# Autodesk Inventor assembly: scaffolding
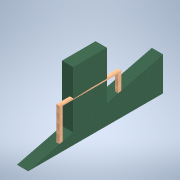
[picture p0: Inventor's stored thumbnail of the model, 180x180]
Saved by Autodesk Inventor 2020.2 (Build 242310000, 310)
## iProperties
Created: 2020-03-28
Part Number: scaffolding
Document SubType Name: Assembly
Designer: robst
Author: robst
## Documents named in this file (5)
- C:\git\CAD-Development\robSteele\HouseProjects\RoofChimney\scaffolding.iam
- C:\git\CAD-Development\robSteele\HouseProjects\RoofChimney\roof.ipt
- C:\git\CAD-Development\robSteele\HouseProjects\RoofChimney\4x4x18-post.ipt
- C:\git\CAD-Development\robSteele\HouseProjects\RoofChimney\2x4x66-board.ipt
- C:\git\CAD-Development\robSteele\HouseProjects\RoofChimney\4x4x33-5_8-post.ipt
## Components (4 placed, 4 different names)
1. roof:1 — Mate:1, Flush:1, Flush:2, Mate:3, Flush:5
2. 4x4x18-post:1 — Mate:1, Flush:1, Flush:2, Mate:2, Flush:3, Flush:4
3. 2x4x66-board:1 — Mate:2, Flush:3, Flush:4, Flush:6
4. 4x4x33-5_8-post:1 — Mate:3, Flush:5, Flush:6
## Relationships (9: Flush 6, Mate 3)
- Mate:1: roof:1 ↔ 4x4x18-post:1
- Flush:1: roof:1 ↔ 4x4x18-post:1
- Flush:2 (1130.3 mm): roof:1 ↔ 4x4x18-post:1
- Mate:2: 4x4x18-post:1 ↔ 2x4x66-board:1
- Flush:3: 4x4x18-post:1 ↔ 2x4x66-board:1
- Flush:4: 4x4x18-post:1 ↔ 2x4x66-board:1
- Mate:3: roof:1 ↔ 4x4x33-5_8-post:1
- Flush:5: roof:1 ↔ 4x4x33-5_8-post:1
- Flush:6: 2x4x66-board:1 ↔ 4x4x33-5_8-post:1
